# Autodesk Inventor assembly: Tanque5G
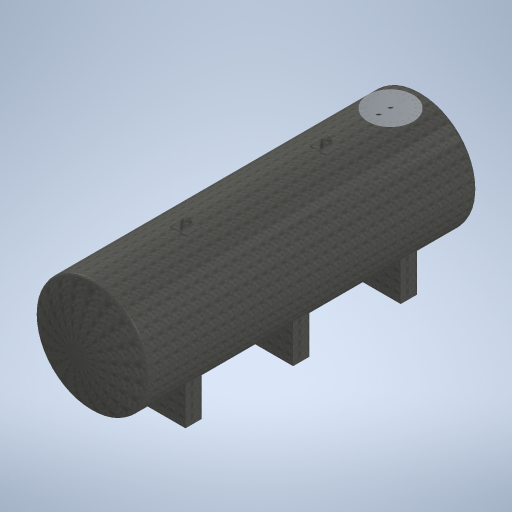
[picture p0: Inventor's stored thumbnail of the model, 512x512]
Saved by Autodesk Inventor 2023 (Build 270158000, 158)
## iProperties
RuleStatus: InUse
Created: 2022-11-02
Part Number: Tanque5G
Document SubType Name: Assembly
Designer: Juanse
AfterAnyUserParamChange0: Actualiza
Author: Juanse
## Documents named in this file (9)
- F:\Alejandro\proyecto comp\Tanque_Parametrizado (2)\Tanque_Parametrizado\Workspaces\Workspace\Tanque5G.iam
- F:\Alejandro\proyecto comp\Tanque_Parametrizado (2)\Tanque_Parametrizado\Workspaces\Workspace\Tanque5000.ipt
- F:\Alejandro\proyecto comp\Tanque_Parametrizado (2)\Tanque_Parametrizado\Workspaces\Workspace\Brida_cuello_tapa.ipt
- F:\Alejandro\proyecto comp\Tanque_Parametrizado (2)\Tanque_Parametrizado\Workspaces\Workspace\Tapa1.ipt
- F:\Alejandro\proyecto comp\Tanque_Parametrizado (2)\Tanque_Parametrizado\Workspaces\Workspace\Tapa2.ipt
- F:\Alejandro\proyecto comp\Tanque_Parametrizado (2)\Tanque_Parametrizado\Libraries\Content Center Files\en-US\ANSI B18.22.1\ANSI B18.22.1 - 1_2 - wide - Type A.ipt
- F:\Alejandro\proyecto comp\Tanque_Parametrizado (2)\Tanque_Parametrizado\Libraries\Content Center Files\en-US\IFI 111\IFI 111 - 1_2-13 UNC x 1,25.ipt
- F:\Alejandro\proyecto comp\Tanque_Parametrizado (2)\Tanque_Parametrizado\Libraries\Content Center Files\en-US\AS 2465(3)\AS 2465 - 1_2  UNC(2).ipt
- F:\Alejandro\proyecto comp\Tanque_Parametrizado (2)\Tanque_Parametrizado\Libraries\Content Center Files\en-US\ASTM F436(1)\ASTM F436 - 1_2(1).ipt
## Components (196 placed, 8 different names)
1. Tanque5000:1 — Mate:1, Flush:3, Mate:3, Mate:4, Mate:6
2. Brida_cuello_tapa:1 — Mate:4, Mate:5, Mate:6, Mate:7, Mate:8, Mate:9, Mate:10, Mate:11, Mate:12, Mate:13, Mate:14, Mate:16, Mate:17
3. Tapa1:1 — Mate:7, Mate:8, Mate:9, Mate:15, Mate:18, Mate:19, Mate:20
4. Tapa2:1 — Mate:10, Mate:11, Mate:12
5. AS 2465 (Unified hexagon bolts, screws and nuts (UNC and UNF threads) - Inch 1/2  UNC:1 — Insert:3
6. Plain Washer (Inch) 1/2 - wide - Type A:1 — Mate:13, Mate:14, Insert:1
7. Circular Washer (Inch) 1/2:1 — Mate:17, Mate:18, Insert:3
8. Plain Washer (Inch) 1/2 - wide - Type A:2 — Mate:15, Mate:16, Insert:2
9. Hex Flange Screw - Inch (IFI) 1/2-13 UNC x 1,25:2 — Insert:2
10. Circular Washer (Inch) 1/2:2 — Mate:19, Mate:20, Insert:4
11. AS 2465 (Unified hexagon bolts, screws and nuts (UNC and UNF threads) - Inch 1/2  UNC:2 — Insert:4
12. Hex Flange Screw - Inch (IFI) 1/2-13 UNC x 1,25:1 — Insert:1
13. AS 2465 (Unified hexagon bolts, screws and nuts (UNC and UNF threads) - Inch 1/2  UNC:3
14. Plain Washer (Inch) 1/2 - wide - Type A:3
15. Circular Washer (Inch) 1/2:3
16. Plain Washer (Inch) 1/2 - wide - Type A:4
17. Hex Flange Screw - Inch (IFI) 1/2-13 UNC x 1,25:3
18. Circular Washer (Inch) 1/2:4
19. AS 2465 (Unified hexagon bolts, screws and nuts (UNC and UNF threads) - Inch 1/2  UNC:4
20. Hex Flange Screw - Inch (IFI) 1/2-13 UNC x 1,25:4
21. AS 2465 (Unified hexagon bolts, screws and nuts (UNC and UNF threads) - Inch 1/2  UNC:5
22. Plain Washer (Inch) 1/2 - wide - Type A:5
23. Circular Washer (Inch) 1/2:5
24. Plain Washer (Inch) 1/2 - wide - Type A:6
25. Hex Flange Screw - Inch (IFI) 1/2-13 UNC x 1,25:5
26. Circular Washer (Inch) 1/2:6
27. AS 2465 (Unified hexagon bolts, screws and nuts (UNC and UNF threads) - Inch 1/2  UNC:6
28. Hex Flange Screw - Inch (IFI) 1/2-13 UNC x 1,25:6
29. AS 2465 (Unified hexagon bolts, screws and nuts (UNC and UNF threads) - Inch 1/2  UNC:7
30. Plain Washer (Inch) 1/2 - wide - Type A:7
31. Circular Washer (Inch) 1/2:7
32. Plain Washer (Inch) 1/2 - wide - Type A:8
33. Hex Flange Screw - Inch (IFI) 1/2-13 UNC x 1,25:7
34. Circular Washer (Inch) 1/2:8
35. AS 2465 (Unified hexagon bolts, screws and nuts (UNC and UNF threads) - Inch 1/2  UNC:8
36. Hex Flange Screw - Inch (IFI) 1/2-13 UNC x 1,25:8
37. AS 2465 (Unified hexagon bolts, screws and nuts (UNC and UNF threads) - Inch 1/2  UNC:9
38. Plain Washer (Inch) 1/2 - wide - Type A:9
39. Circular Washer (Inch) 1/2:9
40. Plain Washer (Inch) 1/2 - wide - Type A:10
41. Hex Flange Screw - Inch (IFI) 1/2-13 UNC x 1,25:9
42. Circular Washer (Inch) 1/2:10
43. AS 2465 (Unified hexagon bolts, screws and nuts (UNC and UNF threads) - Inch 1/2  UNC:10
44. Hex Flange Screw - Inch (IFI) 1/2-13 UNC x 1,25:10
45. AS 2465 (Unified hexagon bolts, screws and nuts (UNC and UNF threads) - Inch 1/2  UNC:11
46. Plain Washer (Inch) 1/2 - wide - Type A:11
47. Circular Washer (Inch) 1/2:11
48. Plain Washer (Inch) 1/2 - wide - Type A:12
49. Hex Flange Screw - Inch (IFI) 1/2-13 UNC x 1,25:11
50. Circular Washer (Inch) 1/2:12
51. AS 2465 (Unified hexagon bolts, screws and nuts (UNC and UNF threads) - Inch 1/2  UNC:12
52. Hex Flange Screw - Inch (IFI) 1/2-13 UNC x 1,25:12
53. AS 2465 (Unified hexagon bolts, screws and nuts (UNC and UNF threads) - Inch 1/2  UNC:13
54. Plain Washer (Inch) 1/2 - wide - Type A:13
55. Circular Washer (Inch) 1/2:13
56. Plain Washer (Inch) 1/2 - wide - Type A:14
57. Hex Flange Screw - Inch (IFI) 1/2-13 UNC x 1,25:13
58. Circular Washer (Inch) 1/2:14
59. AS 2465 (Unified hexagon bolts, screws and nuts (UNC and UNF threads) - Inch 1/2  UNC:14
60. Hex Flange Screw - Inch (IFI) 1/2-13 UNC x 1,25:14
61. AS 2465 (Unified hexagon bolts, screws and nuts (UNC and UNF threads) - Inch 1/2  UNC:15
62. Plain Washer (Inch) 1/2 - wide - Type A:15
63. Circular Washer (Inch) 1/2:15
64. Plain Washer (Inch) 1/2 - wide - Type A:16
65. Hex Flange Screw - Inch (IFI) 1/2-13 UNC x 1,25:15
66. Circular Washer (Inch) 1/2:16
67. AS 2465 (Unified hexagon bolts, screws and nuts (UNC and UNF threads) - Inch 1/2  UNC:16
68. Hex Flange Screw - Inch (IFI) 1/2-13 UNC x 1,25:16
69. AS 2465 (Unified hexagon bolts, screws and nuts (UNC and UNF threads) - Inch 1/2  UNC:17
70. Plain Washer (Inch) 1/2 - wide - Type A:17
71. Circular Washer (Inch) 1/2:17
72. Plain Washer (Inch) 1/2 - wide - Type A:18
73. Hex Flange Screw - Inch (IFI) 1/2-13 UNC x 1,25:17
74. Circular Washer (Inch) 1/2:18
75. AS 2465 (Unified hexagon bolts, screws and nuts (UNC and UNF threads) - Inch 1/2  UNC:18
76. Hex Flange Screw - Inch (IFI) 1/2-13 UNC x 1,25:18
77. AS 2465 (Unified hexagon bolts, screws and nuts (UNC and UNF threads) - Inch 1/2  UNC:19
78. Plain Washer (Inch) 1/2 - wide - Type A:19
79. Circular Washer (Inch) 1/2:19
80. Plain Washer (Inch) 1/2 - wide - Type A:20
81. Hex Flange Screw - Inch (IFI) 1/2-13 UNC x 1,25:19
82. Circular Washer (Inch) 1/2:20
83. AS 2465 (Unified hexagon bolts, screws and nuts (UNC and UNF threads) - Inch 1/2  UNC:20
84. Hex Flange Screw - Inch (IFI) 1/2-13 UNC x 1,25:20
85. AS 2465 (Unified hexagon bolts, screws and nuts (UNC and UNF threads) - Inch 1/2  UNC:21
86. Plain Washer (Inch) 1/2 - wide - Type A:21
87. Circular Washer (Inch) 1/2:21
88. Plain Washer (Inch) 1/2 - wide - Type A:22
89. Hex Flange Screw - Inch (IFI) 1/2-13 UNC x 1,25:21
90. Circular Washer (Inch) 1/2:22
91. AS 2465 (Unified hexagon bolts, screws and nuts (UNC and UNF threads) - Inch 1/2  UNC:22
92. Hex Flange Screw - Inch (IFI) 1/2-13 UNC x 1,25:22
93. AS 2465 (Unified hexagon bolts, screws and nuts (UNC and UNF threads) - Inch 1/2  UNC:23
94. Plain Washer (Inch) 1/2 - wide - Type A:23
95. Circular Washer (Inch) 1/2:23
96. Plain Washer (Inch) 1/2 - wide - Type A:24
97. Hex Flange Screw - Inch (IFI) 1/2-13 UNC x 1,25:23
98. Circular Washer (Inch) 1/2:24
99. AS 2465 (Unified hexagon bolts, screws and nuts (UNC and UNF threads) - Inch 1/2  UNC:24
100. Hex Flange Screw - Inch (IFI) 1/2-13 UNC x 1,25:24
101. AS 2465 (Unified hexagon bolts, screws and nuts (UNC and UNF threads) - Inch 1/2  UNC:25
102. Plain Washer (Inch) 1/2 - wide - Type A:25
103. Circular Washer (Inch) 1/2:25
104. Plain Washer (Inch) 1/2 - wide - Type A:26
105. Hex Flange Screw - Inch (IFI) 1/2-13 UNC x 1,25:25
106. Circular Washer (Inch) 1/2:26
107. AS 2465 (Unified hexagon bolts, screws and nuts (UNC and UNF threads) - Inch 1/2  UNC:26
108. Hex Flange Screw - Inch (IFI) 1/2-13 UNC x 1,25:26
109. AS 2465 (Unified hexagon bolts, screws and nuts (UNC and UNF threads) - Inch 1/2  UNC:27
110. Plain Washer (Inch) 1/2 - wide - Type A:27
111. Circular Washer (Inch) 1/2:27
112. Plain Washer (Inch) 1/2 - wide - Type A:28
113. Hex Flange Screw - Inch (IFI) 1/2-13 UNC x 1,25:27
114. Circular Washer (Inch) 1/2:28
115. AS 2465 (Unified hexagon bolts, screws and nuts (UNC and UNF threads) - Inch 1/2  UNC:28
116. Hex Flange Screw - Inch (IFI) 1/2-13 UNC x 1,25:28
117. AS 2465 (Unified hexagon bolts, screws and nuts (UNC and UNF threads) - Inch 1/2  UNC:29
118. Plain Washer (Inch) 1/2 - wide - Type A:29
119. Circular Washer (Inch) 1/2:29
120. Plain Washer (Inch) 1/2 - wide - Type A:30
121. Hex Flange Screw - Inch (IFI) 1/2-13 UNC x 1,25:29
122. Circular Washer (Inch) 1/2:30
123. AS 2465 (Unified hexagon bolts, screws and nuts (UNC and UNF threads) - Inch 1/2  UNC:30
124. Hex Flange Screw - Inch (IFI) 1/2-13 UNC x 1,25:30
125. AS 2465 (Unified hexagon bolts, screws and nuts (UNC and UNF threads) - Inch 1/2  UNC:31
126. Plain Washer (Inch) 1/2 - wide - Type A:31
127. Circular Washer (Inch) 1/2:31
128. Plain Washer (Inch) 1/2 - wide - Type A:32
129. Hex Flange Screw - Inch (IFI) 1/2-13 UNC x 1,25:31
130. Circular Washer (Inch) 1/2:32
131. AS 2465 (Unified hexagon bolts, screws and nuts (UNC and UNF threads) - Inch 1/2  UNC:32
132. Hex Flange Screw - Inch (IFI) 1/2-13 UNC x 1,25:32
133. AS 2465 (Unified hexagon bolts, screws and nuts (UNC and UNF threads) - Inch 1/2  UNC:33
134. Plain Washer (Inch) 1/2 - wide - Type A:33
135. Circular Washer (Inch) 1/2:33
136. Plain Washer (Inch) 1/2 - wide - Type A:34
137. Hex Flange Screw - Inch (IFI) 1/2-13 UNC x 1,25:33
138. Circular Washer (Inch) 1/2:34
139. AS 2465 (Unified hexagon bolts, screws and nuts (UNC and UNF threads) - Inch 1/2  UNC:34
140. Hex Flange Screw - Inch (IFI) 1/2-13 UNC x 1,25:34
141. AS 2465 (Unified hexagon bolts, screws and nuts (UNC and UNF threads) - Inch 1/2  UNC:35
142. Plain Washer (Inch) 1/2 - wide - Type A:35
143. Circular Washer (Inch) 1/2:35
144. Plain Washer (Inch) 1/2 - wide - Type A:36
145. Hex Flange Screw - Inch (IFI) 1/2-13 UNC x 1,25:35
146. Circular Washer (Inch) 1/2:36
147. AS 2465 (Unified hexagon bolts, screws and nuts (UNC and UNF threads) - Inch 1/2  UNC:36
148. Hex Flange Screw - Inch (IFI) 1/2-13 UNC x 1,25:36
149. AS 2465 (Unified hexagon bolts, screws and nuts (UNC and UNF threads) - Inch 1/2  UNC:37
150. Plain Washer (Inch) 1/2 - wide - Type A:37
151. Circular Washer (Inch) 1/2:37
152. Plain Washer (Inch) 1/2 - wide - Type A:38
153. Hex Flange Screw - Inch (IFI) 1/2-13 UNC x 1,25:37
154. Circular Washer (Inch) 1/2:38
155. AS 2465 (Unified hexagon bolts, screws and nuts (UNC and UNF threads) - Inch 1/2  UNC:38
156. Hex Flange Screw - Inch (IFI) 1/2-13 UNC x 1,25:38
157. AS 2465 (Unified hexagon bolts, screws and nuts (UNC and UNF threads) - Inch 1/2  UNC:39
158. Plain Washer (Inch) 1/2 - wide - Type A:39
159. Circular Washer (Inch) 1/2:39
160. Plain Washer (Inch) 1/2 - wide - Type A:40
161. Hex Flange Screw - Inch (IFI) 1/2-13 UNC x 1,25:39
162. Circular Washer (Inch) 1/2:40
163. AS 2465 (Unified hexagon bolts, screws and nuts (UNC and UNF threads) - Inch 1/2  UNC:40
164. Hex Flange Screw - Inch (IFI) 1/2-13 UNC x 1,25:40
165. AS 2465 (Unified hexagon bolts, screws and nuts (UNC and UNF threads) - Inch 1/2  UNC:41
166. Plain Washer (Inch) 1/2 - wide - Type A:41
167. Circular Washer (Inch) 1/2:41
168. Plain Washer (Inch) 1/2 - wide - Type A:42
169. Hex Flange Screw - Inch (IFI) 1/2-13 UNC x 1,25:41
170. Circular Washer (Inch) 1/2:42
171. AS 2465 (Unified hexagon bolts, screws and nuts (UNC and UNF threads) - Inch 1/2  UNC:42
172. Hex Flange Screw - Inch (IFI) 1/2-13 UNC x 1,25:42
173. AS 2465 (Unified hexagon bolts, screws and nuts (UNC and UNF threads) - Inch 1/2  UNC:43
174. Plain Washer (Inch) 1/2 - wide - Type A:43
175. Circular Washer (Inch) 1/2:43
176. Plain Washer (Inch) 1/2 - wide - Type A:44
177. Hex Flange Screw - Inch (IFI) 1/2-13 UNC x 1,25:43
178. Circular Washer (Inch) 1/2:44
179. AS 2465 (Unified hexagon bolts, screws and nuts (UNC and UNF threads) - Inch 1/2  UNC:44
180. Hex Flange Screw - Inch (IFI) 1/2-13 UNC x 1,25:44
181. AS 2465 (Unified hexagon bolts, screws and nuts (UNC and UNF threads) - Inch 1/2  UNC:45
182. Plain Washer (Inch) 1/2 - wide - Type A:45
183. Circular Washer (Inch) 1/2:45
184. Plain Washer (Inch) 1/2 - wide - Type A:46
185. Hex Flange Screw - Inch (IFI) 1/2-13 UNC x 1,25:45
186. Circular Washer (Inch) 1/2:46
187. AS 2465 (Unified hexagon bolts, screws and nuts (UNC and UNF threads) - Inch 1/2  UNC:46
188. Hex Flange Screw - Inch (IFI) 1/2-13 UNC x 1,25:46
189. AS 2465 (Unified hexagon bolts, screws and nuts (UNC and UNF threads) - Inch 1/2  UNC:47
190. Plain Washer (Inch) 1/2 - wide - Type A:47
191. Circular Washer (Inch) 1/2:47
192. Plain Washer (Inch) 1/2 - wide - Type A:48
193. Hex Flange Screw - Inch (IFI) 1/2-13 UNC x 1,25:47
194. Circular Washer (Inch) 1/2:48
195. AS 2465 (Unified hexagon bolts, screws and nuts (UNC and UNF threads) - Inch 1/2  UNC:48
196. Hex Flange Screw - Inch (IFI) 1/2-13 UNC x 1,25:48
## Component patterns: (24 elements, first: AS 2465 (Unified hexagon bolts, screws and nuts (UNC and UNF threads) - Inch 1/2  UNC:1 + Plain Washer (Inch) 1/2 - wide - Type A:1 + Circular Washer (Inch) 1/2:1 + Plain Washer (Inch) 1/2 - wide - Type A:2 + Hex Flange Screw - Inch (IFI) 1/2-13 UNC x 1,25:2 + Circular Washer (Inch) 1/2:2 + AS 2465 (Unified hexagon bolts, screws and nuts (UNC and UNF threads) - Inch 1/2  UNC:2 + Hex Flange Screw - Inch (IFI) 1/2-13 UNC x 1,25:1)
## Relationships (24: Mate 19, Insert 4, Flush 1)
- Mate:1: Tanque5000:1
- Flush:3: Tanque5000:1
- Mate:3: Tanque5000:1
- Mate:4: Tanque5000:1 ↔ Brida_cuello_tapa:1
- Mate:5: Brida_cuello_tapa:1
- Mate:6: Tanque5000:1 ↔ Brida_cuello_tapa:1
- Mate:7: Brida_cuello_tapa:1 ↔ Tapa1:1
- Mate:8: Brida_cuello_tapa:1 ↔ Tapa1:1
- Mate:9: Brida_cuello_tapa:1 ↔ Tapa1:1
- Mate:10: Brida_cuello_tapa:1 ↔ Tapa2:1
- Mate:11: Brida_cuello_tapa:1 ↔ Tapa2:1
- Mate:12: Brida_cuello_tapa:1 ↔ Tapa2:1
- Mate:13: Brida_cuello_tapa:1 ↔ Plain Washer (Inch) 1/2 - wide - Type A:1
- Mate:14: Brida_cuello_tapa:1 ↔ Plain Washer (Inch) 1/2 - wide - Type A:1
- Mate:15: Tapa1:1 ↔ Plain Washer (Inch) 1/2 - wide - Type A:2
- Mate:16: Brida_cuello_tapa:1 ↔ Plain Washer (Inch) 1/2 - wide - Type A:2
- Insert:1: Plain Washer (Inch) 1/2 - wide - Type A:1 ↔ Hex Flange Screw - Inch (IFI) 1/2-13 UNC x 1,25:1
- Insert:2: Plain Washer (Inch) 1/2 - wide - Type A:2 ↔ Hex Flange Screw - Inch (IFI) 1/2-13 UNC x 1,25:2
- Mate:17: Brida_cuello_tapa:1 ↔ Circular Washer (Inch) 1/2:1
- Mate:18: Tapa1:1 ↔ Circular Washer (Inch) 1/2:1
- Mate:19: Tapa1:1 ↔ Circular Washer (Inch) 1/2:2
- Mate:20: Tapa1:1 ↔ Circular Washer (Inch) 1/2:2
- Insert:3: AS 2465 (Unified hexagon bolts, screws and nuts (UNC and UNF threads) - Inch 1/2  UNC:1 ↔ Circular Washer (Inch) 1/2:1
- Insert:4: Circular Washer (Inch) 1/2:2 ↔ AS 2465 (Unified hexagon bolts, screws and nuts (UNC and UNF threads) - Inch 1/2  UNC:2
